# Autodesk Inventor assembly: assembled_rack
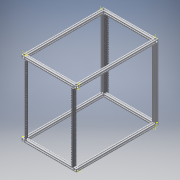
[picture p0: Inventor's stored thumbnail of the model, 180x180]
Saved by Autodesk Inventor 2016 (Build 200138000, 138)
## iProperties
Created: 2016-10-05
Part Number: assembled_rack
Document SubType Name: Assembly
Designer: gmmar
Author: gmmar
## Documents named in this file (6)
- C:\Users\gmmar\AppData\Local\lxss\home\marco\rack-design\parts\assembled_rack.iam
- C:\Users\gmmar\AppData\Local\lxss\home\marco\rack-design\parts\30x30_extrude_horizontal_750mm.ipt
- C:\Users\gmmar\AppData\Local\lxss\home\marco\rack-design\parts\30x30_3way_cubic_con.ipt
- C:\Users\gmmar\AppData\Local\lxss\home\marco\rack-design\parts\30x30_extrude_horizontal_481mm.ipt
- C:\Users\gmmar\AppData\Local\lxss\home\marco\rack-design\parts\30x30_extrude_vertical_680mm.ipt
- C:\Users\gmmar\AppData\Local\lxss\home\marco\rack-design\parts\15U_rack_strip.ipt
## Components (24 placed, 5 different names)
1. 30x30_3way_cubic_con:1 — Mate:1, Mate:5, Mate:29
2. 30x30_extrude_horizontal_481mm:1 — Mate:1, Mate:2, Mate:3
3. 30x30_3way_cubic_con:2 — Mate:2, Mate:3, Mate:4, Mate:8, Mate:30
4. 30x30_extrude_vertical_680mm:1 — Mate:4, Mate:6, Mate:7, Mate:8, Mate:12
5. 30x30_extrude_vertical_680mm:2 — Mate:5, Mate:14, Mate:17
6. 30x30_3way_cubic_con:3 — Mate:6, Mate:7, Mate:9, Mate:10, Mate:19
7. 30x30_extrude_horizontal_481mm:2 — Mate:9, Mate:10, Mate:11, Mate:13, Flush:1, Flush:2, Mate:15, Mate:16
8. 15U_rack_strip:1 — Mate:11, Mate:12, Flush:2
9. 15U_rack_strip:2 — Mate:13, Flush:1, Mate:14
10. 30x30_3way_cubic_con:4 — Mate:15, Mate:16, Mate:17, Mate:18
11. 30x30_extrude_horizontal_750mm:1 — Mate:19, Flush:3
12. 30x30_extrude_horizontal_750mm:2 — Mate:18, Mate:20, Mate:21
13. 30x30_3way_cubic_con:5 — Mate:20, Mate:21, Mate:24
14. 30x30_3way_cubic_con:6 — Flush:3, Mate:22, Mate:23
15. 30x30_extrude_horizontal_481mm:3 — Mate:22, Mate:25, Flush:4, Mate:27, Flush:5
16. 30x30_extrude_vertical_680mm:3 — Mate:23, Mate:26, Flush:11
17. 30x30_extrude_vertical_680mm:4 — Mate:24, Mate:28, Flush:8
18. 15U_rack_strip:3 — Mate:25, Flush:4, Mate:26
19. 15U_rack_strip:4 — Mate:27, Flush:5, Mate:28
20. 30x30_extrude_horizontal_750mm:3 — Mate:29, Flush:6, Mate:31, Flush:7
21. 30x30_extrude_horizontal_750mm:4 — Mate:30, Flush:10
22. 30x30_3way_cubic_con:7 — Flush:10, Flush:11, Mate:32
23. 30x30_3way_cubic_con:8 — Flush:6, Mate:31, Flush:7, Flush:8, Flush:12
24. 30x30_extrude_horizontal_481mm:4 — Mate:32, Flush:12
## Relationships (43: Mate 32, Flush 11)
- Mate:1: 30x30_3way_cubic_con:1 ↔ 30x30_extrude_horizontal_481mm:1
- Mate:2: 30x30_extrude_horizontal_481mm:1 ↔ 30x30_3way_cubic_con:2
- Mate:3: 30x30_extrude_horizontal_481mm:1 ↔ 30x30_3way_cubic_con:2
- Mate:4: 30x30_3way_cubic_con:2 ↔ 30x30_extrude_vertical_680mm:1
- Mate:5: 30x30_3way_cubic_con:1 ↔ 30x30_extrude_vertical_680mm:2
- Mate:6: 30x30_extrude_vertical_680mm:1 ↔ 30x30_3way_cubic_con:3
- Mate:7: 30x30_extrude_vertical_680mm:1 ↔ 30x30_3way_cubic_con:3
- Mate:8: 30x30_3way_cubic_con:2 ↔ 30x30_extrude_vertical_680mm:1
- Mate:9: 30x30_3way_cubic_con:3 ↔ 30x30_extrude_horizontal_481mm:2
- Mate:10: 30x30_3way_cubic_con:3 ↔ 30x30_extrude_horizontal_481mm:2
- Mate:11: 30x30_extrude_horizontal_481mm:2 ↔ 15U_rack_strip:1
- Mate:12: 30x30_extrude_vertical_680mm:1 ↔ 15U_rack_strip:1
- Mate:13: 30x30_extrude_horizontal_481mm:2 ↔ 15U_rack_strip:2
- Flush:1: 30x30_extrude_horizontal_481mm:2 ↔ 15U_rack_strip:2
- Mate:14: 30x30_extrude_vertical_680mm:2 ↔ 15U_rack_strip:2
- Flush:2: 30x30_extrude_horizontal_481mm:2 ↔ 15U_rack_strip:1
- Mate:15: 30x30_extrude_horizontal_481mm:2 ↔ 30x30_3way_cubic_con:4
- Mate:16: 30x30_extrude_horizontal_481mm:2 ↔ 30x30_3way_cubic_con:4
- Mate:17: 30x30_extrude_vertical_680mm:2 ↔ 30x30_3way_cubic_con:4
- Mate:18: 30x30_3way_cubic_con:4 ↔ 30x30_extrude_horizontal_750mm:2
- Mate:19: 30x30_3way_cubic_con:3 ↔ 30x30_extrude_horizontal_750mm:1
- Mate:20: 30x30_extrude_horizontal_750mm:2 ↔ 30x30_3way_cubic_con:5
- Mate:21: 30x30_extrude_horizontal_750mm:2 ↔ 30x30_3way_cubic_con:5
- Flush:3: 30x30_extrude_horizontal_750mm:1 ↔ 30x30_3way_cubic_con:6
- Mate:22: 30x30_3way_cubic_con:6 ↔ 30x30_extrude_horizontal_481mm:3
- Mate:23: 30x30_3way_cubic_con:6 ↔ 30x30_extrude_vertical_680mm:3
- Mate:24: 30x30_3way_cubic_con:5 ↔ 30x30_extrude_vertical_680mm:4
- Mate:25: 30x30_extrude_horizontal_481mm:3 ↔ 15U_rack_strip:3
- Flush:4: 30x30_extrude_horizontal_481mm:3 ↔ 15U_rack_strip:3
- Mate:26: 30x30_extrude_vertical_680mm:3 ↔ 15U_rack_strip:3
- Mate:27: 30x30_extrude_horizontal_481mm:3 ↔ 15U_rack_strip:4
- Flush:5: 30x30_extrude_horizontal_481mm:3 ↔ 15U_rack_strip:4
- Mate:28: 30x30_extrude_vertical_680mm:4 ↔ 15U_rack_strip:4
- Mate:29: 30x30_3way_cubic_con:1 ↔ 30x30_extrude_horizontal_750mm:3
- Mate:30: 30x30_3way_cubic_con:2 ↔ 30x30_extrude_horizontal_750mm:4
- Flush:6: 30x30_extrude_horizontal_750mm:3 ↔ 30x30_3way_cubic_con:8
- Mate:31: 30x30_extrude_horizontal_750mm:3 ↔ 30x30_3way_cubic_con:8
- Flush:7: 30x30_extrude_horizontal_750mm:3 ↔ 30x30_3way_cubic_con:8
- Flush:8: 30x30_extrude_vertical_680mm:4 ↔ 30x30_3way_cubic_con:8
- Flush:10: 30x30_extrude_horizontal_750mm:4 ↔ 30x30_3way_cubic_con:7
- Flush:11: 30x30_extrude_vertical_680mm:3 ↔ 30x30_3way_cubic_con:7
- Mate:32: 30x30_3way_cubic_con:7 ↔ 30x30_extrude_horizontal_481mm:4
- Flush:12: 30x30_3way_cubic_con:8 ↔ 30x30_extrude_horizontal_481mm:4
